# Autodesk Inventor assembly: TB_MAIN_A_001
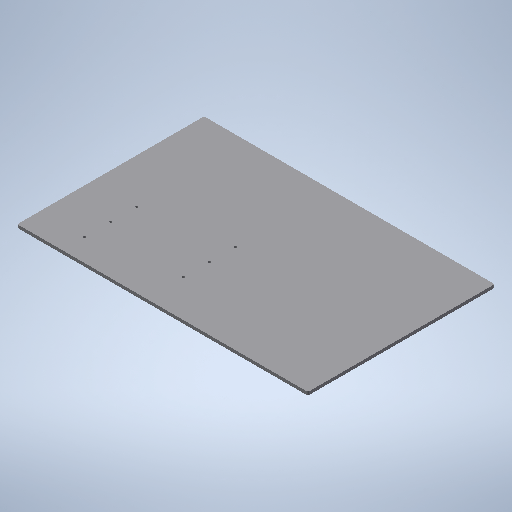
[picture p0: Inventor's stored thumbnail of the model, 512x512]
Saved by Autodesk Inventor 2025.4 (Build 294407000, 407)
## iProperties
Created: 2026-07-01
Part Number: TB_MAIN_A_001
Document SubType Name: Assembly
Designer: louis
Author: louis
## Documents named in this file (2)
- C:\Users\louis\OneDrive\Desktop\R_Trident\02_CAD\05_Top_Assembly\TB_MAIN_A_001.iam
- C:\Users\louis\OneDrive\Desktop\R_Trident\02_CAD\03_Parts_Custom\TB_FRM_MC_001_BasePlate.ipt
## Components (1 placed, 1 different names)
1. TB_FRM_MC_001_BasePlate:1 — Flush:1, Flush:2, Flush:3
## Relationships (3: Flush 3)
- Flush:1: TB_FRM_MC_001_BasePlate:1
- Flush:2: TB_FRM_MC_001_BasePlate:1
- Flush:3: TB_FRM_MC_001_BasePlate:1
